# Autodesk Inventor assembly: MMAE 232 Sustainalble Chair V2- Nicholas Skiba
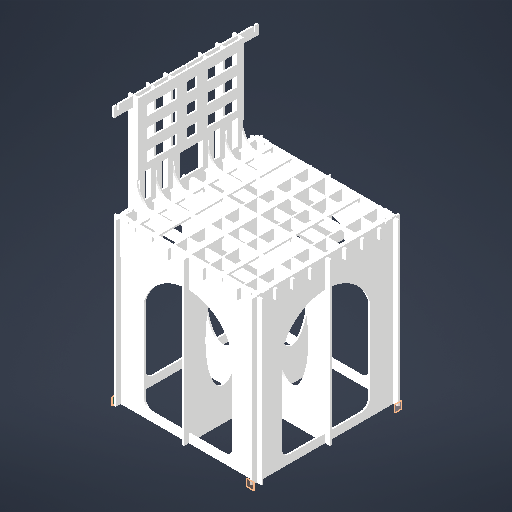
[picture p0: Inventor's stored thumbnail of the model, 512x512]
Saved by Autodesk Inventor 2027.1 (Build 311270010, 270A)
## iProperties
Created: 2025-09-21
Part Number: MMAE 232 Sustainalble Chair V2- Nicholas Skiba
Document SubType Name: Assembly
Designer: Nick
Mass: 788.264 g
Surface Area: 24924.6 cm^2
Volume: 5551.23 cm^3
Density: 0.141998 g/cm^3
Author: Nick
## Documents named in this file (10)
- C:\Users\Nick\Desktop\Important\Github\Sustainable-Chair\CAD\sustainable_chair_assembly.iam
- C:\Users\Nick\Desktop\Important\Github\Sustainable-Chair\CAD\Parts\inside_leg_2.ipt
- C:\Users\Nick\Desktop\Important\Github\Sustainable-Chair\CAD\Parts\inside_leg.ipt
- C:\Users\Nick\Desktop\Important\Github\Sustainable-Chair\CAD\Parts\outside_leg.ipt
- C:\Users\Nick\Desktop\Important\Github\Sustainable-Chair\CAD\Parts\slats_back_under.ipt
- C:\Users\Nick\Desktop\Important\Github\Sustainable-Chair\CAD\Parts\slats.ipt
- C:\Users\Nick\Desktop\Important\Github\Sustainable-Chair\CAD\Parts\slats_back_over.ipt
- C:\Users\Nick\Desktop\Important\Github\Sustainable-Chair\CAD\Parts\seat.ipt
- C:\Users\Nick\Desktop\Important\Github\Sustainable-Chair\CAD\Parts\slats_under.ipt
- C:\Users\Nick\Desktop\Important\Github\Sustainable-Chair\CAD\Parts\backrest.ipt
## Components (18 placed, 9 different names)
1. MMAE 232 Sustainalble Chair Inside Leg2 - Nicholas Skiba:1 — Mate:1, Flush:1, Mate:2, Mate:3, Flush:2, Mate:6, Mate:7, Mate:9, Flush:6, Flush:7, Flush:8
2. MMAE 232 Sustainalble Chair Inside Leg - Nicholas Skiba:1 — Mate:1, Flush:1, Mate:2, Mate:3, Mate:4, Mate:5, Flush:3, Mate:11, Flush:9
3. MMAE 232 Sustainalble Chair Outside Leg - Nicholas Skiba:1 — Mate:4, Flush:2, Mate:5, Mate:8, Mate:10, Flush:10, Mate:13
4. MMAE 232 Sustainalble Chair Outside Leg - Nicholas Skiba:3 — Mate:6, Mate:7, Mate:8, Flush:3, Flush:4, Mate:12, Mate:14
5. MMAE 232 Sustainalble Chair Outside Leg - Nicholas Skiba:4 — Mate:9, Flush:4, Mate:10, Flush:5, Flush:16
6. MMAE 232 Sustainalble Chair Outside Leg - Nicholas Skiba:5 — Flush:5, Flush:6, Mate:11, Flush:17
7. MMAE 232 Sustainalble Chair Slats Under - Nicholas Skiba:1 — Mate:17, Mate:18, Flush:13
8. MMAE 232 Sustainalble Chair Back Rest - Nicholas Skiba:1 — Mate:19, Flush:14, Flush:15
9. MMAE 232 Sustainalble Chair Seat - Nicholas Skiba:1 — Mate:20, Flush:16, Flush:17
10. MMAE 232 Sustainalble Chair Slats - Nicholas Skiba:1 — Flush:9, Flush:10, Mate:13
11. MMAE 232 Sustainalble Chair Slats - Nicholas Skiba:2
12. MMAE 232 Sustainalble Chair Slats - Nicholas Skiba:3
13. MMAE 232 Sustainalble Chair Slats And Back Over - Nicholas Skiba:1 — Mate:14, Flush:11, Flush:12
14. MMAE 232 Sustainalble Chair Slats And Back Over - Nicholas Skiba:2
15. MMAE 232 Sustainalble Chair Slats And Back Under - Nicholas Skiba:1 — Flush:7, Flush:8, Mate:12, Flush:13
16. MMAE 232 Sustainalble Chair Slats And Back Under - Nicholas Skiba:5 — Flush:11, Flush:12, Mate:19, Flush:14, Flush:15
17. MMAE 232 Sustainalble Chair Slats And Back Under - Nicholas Skiba:6 — Mate:17, Mate:20
18. MMAE 232 Sustainalble Chair Slats And Back Under - Nicholas Skiba:7 — Mate:18
## Component patterns: (2 elements), (3 elements, first: MMAE 232 Sustainalble Chair Slats - Nicholas Skiba:1), (2 elements, first: MMAE 232 Sustainalble Chair Slats And Back Over - Nicholas Skiba:1), (2 elements, first: MMAE 232 Sustainalble Chair Slats And Back Under - Nicholas Skiba:1), Component Pattern 3:2 (2 elements)
## Relationships (35: Mate 18, Flush 17)
- Mate:1: MMAE 232 Sustainalble Chair Inside Leg2 - Nicholas Skiba:1 ↔ MMAE 232 Sustainalble Chair Inside Leg - Nicholas Skiba:1
- Flush:1: MMAE 232 Sustainalble Chair Inside Leg2 - Nicholas Skiba:1 ↔ MMAE 232 Sustainalble Chair Inside Leg - Nicholas Skiba:1
- Mate:2 (-0.25 mm): MMAE 232 Sustainalble Chair Inside Leg2 - Nicholas Skiba:1 ↔ MMAE 232 Sustainalble Chair Inside Leg - Nicholas Skiba:1
- Mate:3 (-0.25 mm): MMAE 232 Sustainalble Chair Inside Leg2 - Nicholas Skiba:1 ↔ MMAE 232 Sustainalble Chair Inside Leg - Nicholas Skiba:1
- Mate:4: MMAE 232 Sustainalble Chair Inside Leg - Nicholas Skiba:1 ↔ MMAE 232 Sustainalble Chair Outside Leg - Nicholas Skiba:1
- Flush:2: MMAE 232 Sustainalble Chair Inside Leg2 - Nicholas Skiba:1 ↔ MMAE 232 Sustainalble Chair Outside Leg - Nicholas Skiba:1
- Mate:5 (-0.25 mm): MMAE 232 Sustainalble Chair Inside Leg - Nicholas Skiba:1 ↔ MMAE 232 Sustainalble Chair Outside Leg - Nicholas Skiba:1
- Mate:6: MMAE 232 Sustainalble Chair Inside Leg2 - Nicholas Skiba:1 ↔ MMAE 232 Sustainalble Chair Outside Leg - Nicholas Skiba:3
- Mate:7 (-0.25 mm): MMAE 232 Sustainalble Chair Inside Leg2 - Nicholas Skiba:1 ↔ MMAE 232 Sustainalble Chair Outside Leg - Nicholas Skiba:3
- Mate:8 (-0.25 mm): MMAE 232 Sustainalble Chair Outside Leg - Nicholas Skiba:1 ↔ MMAE 232 Sustainalble Chair Outside Leg - Nicholas Skiba:3
- Flush:3: MMAE 232 Sustainalble Chair Inside Leg - Nicholas Skiba:1 ↔ MMAE 232 Sustainalble Chair Outside Leg - Nicholas Skiba:3
- Mate:9: MMAE 232 Sustainalble Chair Inside Leg2 - Nicholas Skiba:1 ↔ MMAE 232 Sustainalble Chair Outside Leg - Nicholas Skiba:4
- Flush:4: MMAE 232 Sustainalble Chair Outside Leg - Nicholas Skiba:3 ↔ MMAE 232 Sustainalble Chair Outside Leg - Nicholas Skiba:4
- Mate:10 (-0.25 mm): MMAE 232 Sustainalble Chair Outside Leg - Nicholas Skiba:1 ↔ MMAE 232 Sustainalble Chair Outside Leg - Nicholas Skiba:4
- Flush:5: MMAE 232 Sustainalble Chair Outside Leg - Nicholas Skiba:4 ↔ MMAE 232 Sustainalble Chair Outside Leg - Nicholas Skiba:5
- Flush:6: MMAE 232 Sustainalble Chair Inside Leg2 - Nicholas Skiba:1 ↔ MMAE 232 Sustainalble Chair Outside Leg - Nicholas Skiba:5
- Mate:11 (-0.25 mm): MMAE 232 Sustainalble Chair Inside Leg - Nicholas Skiba:1 ↔ MMAE 232 Sustainalble Chair Outside Leg - Nicholas Skiba:5
- Flush:7 (5 mm): MMAE 232 Sustainalble Chair Inside Leg2 - Nicholas Skiba:1 ↔ MMAE 232 Sustainalble Chair Slats And Back Under - Nicholas Skiba:1
- Flush:8: MMAE 232 Sustainalble Chair Inside Leg2 - Nicholas Skiba:1 ↔ MMAE 232 Sustainalble Chair Slats And Back Under - Nicholas Skiba:1
- Mate:12 (-0.25 mm): MMAE 232 Sustainalble Chair Outside Leg - Nicholas Skiba:3 ↔ MMAE 232 Sustainalble Chair Slats And Back Under - Nicholas Skiba:1
- Flush:9 (5 mm): MMAE 232 Sustainalble Chair Inside Leg - Nicholas Skiba:1 ↔ MMAE 232 Sustainalble Chair Slats - Nicholas Skiba:1
- Flush:10: MMAE 232 Sustainalble Chair Outside Leg - Nicholas Skiba:1 ↔ MMAE 232 Sustainalble Chair Slats - Nicholas Skiba:1
- Mate:13 (-0.25 mm): MMAE 232 Sustainalble Chair Outside Leg - Nicholas Skiba:1 ↔ MMAE 232 Sustainalble Chair Slats - Nicholas Skiba:1
- Mate:14 (-0.25 mm): MMAE 232 Sustainalble Chair Outside Leg - Nicholas Skiba:3 ↔ MMAE 232 Sustainalble Chair Slats And Back Over - Nicholas Skiba:1
- Flush:11: MMAE 232 Sustainalble Chair Slats And Back Over - Nicholas Skiba:1 ↔ MMAE 232 Sustainalble Chair Slats And Back Under - Nicholas Skiba:5
- Flush:12: MMAE 232 Sustainalble Chair Slats And Back Over - Nicholas Skiba:1 ↔ MMAE 232 Sustainalble Chair Slats And Back Under - Nicholas Skiba:5
- Mate:17 (-0.25 mm): MMAE 232 Sustainalble Chair Slats Under - Nicholas Skiba:1 ↔ MMAE 232 Sustainalble Chair Slats And Back Under - Nicholas Skiba:6
- Mate:18 (-0.25 mm): MMAE 232 Sustainalble Chair Slats Under - Nicholas Skiba:1 ↔ MMAE 232 Sustainalble Chair Slats And Back Under - Nicholas Skiba:7
- Flush:13: MMAE 232 Sustainalble Chair Slats Under - Nicholas Skiba:1 ↔ MMAE 232 Sustainalble Chair Slats And Back Under - Nicholas Skiba:1
- Mate:19: MMAE 232 Sustainalble Chair Back Rest - Nicholas Skiba:1 ↔ MMAE 232 Sustainalble Chair Slats And Back Under - Nicholas Skiba:5
- Flush:14: MMAE 232 Sustainalble Chair Back Rest - Nicholas Skiba:1 ↔ MMAE 232 Sustainalble Chair Slats And Back Under - Nicholas Skiba:5
- Flush:15: MMAE 232 Sustainalble Chair Back Rest - Nicholas Skiba:1 ↔ MMAE 232 Sustainalble Chair Slats And Back Under - Nicholas Skiba:5
- Mate:20: MMAE 232 Sustainalble Chair Seat - Nicholas Skiba:1 ↔ MMAE 232 Sustainalble Chair Slats And Back Under - Nicholas Skiba:6
- Flush:16 (-2.5 mm): MMAE 232 Sustainalble Chair Outside Leg - Nicholas Skiba:4 ↔ MMAE 232 Sustainalble Chair Seat - Nicholas Skiba:1
- Flush:17 (-2.5 mm): MMAE 232 Sustainalble Chair Outside Leg - Nicholas Skiba:5 ↔ MMAE 232 Sustainalble Chair Seat - Nicholas Skiba:1
